# Autodesk Inventor assembly: Assembly1_TT
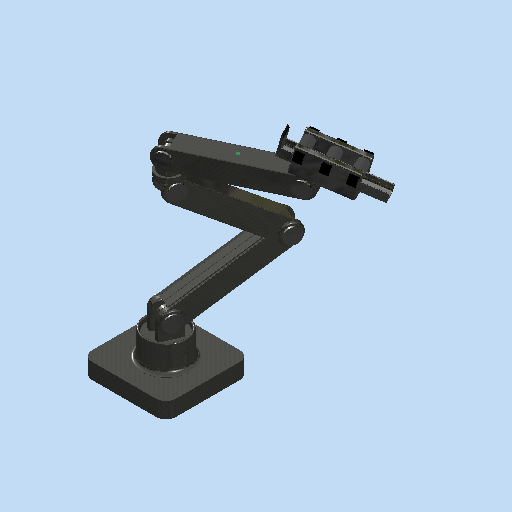
[picture p0: Inventor's stored thumbnail of the model, 512x512]
Saved by Autodesk Inventor 2027.1 (Build 311270010, 270A)
## iProperties
Created: 2026-08-27
Part Number: Assembly1_TT
Document SubType Name: Assembly
Designer: RIDDHIMAN
Author: RIDDHIMAN
## Documents named in this file (12)
- D:\ZINE ROUND 2\Assembly1_TT.iam
- D:\ZINE ROUND 2\HANDBASE2.ipt
- D:\ZINE ROUND 2\TT_ARM1.ipt
- D:\ZINE ROUND 2\TT_ARM12.ipt
- D:\ZINE ROUND 2\HANDBASE1.ipt
- D:\ZINE ROUND 2\joint1.ipt
- D:\ZINE ROUND 2\joint2.ipt
- D:\ZINE ROUND 2\JOINT BASE2.ipt
- D:\ZINE ROUND 2\JOINT BASE1.ipt
- D:\ZINE ROUND 2\SHOOTING GUN.ipt
- D:\ZINE ROUND 2\ROLLER SHAFT.ipt
- D:\ZINE ROUND 2\ROLLER.ipt
## Components (19 placed, 11 different names)
1. HANDBASE2:1 — Rotational:3
2. TT_ARM1:1 — Rotational:1, Rotational:2, Rigid:2
3. TT_ARM12:1 — Rotational:2, Rigid:1, Rigid:3, Rotational:4
4. HANDBASE1:1 — Rotational:1, Rotational:3
5. joint1:1 — Rigid:1
6. joint1:2 — Rigid:2
7. joint2:1 — Rigid:3
8. JOINT BASE2:1 — Rotational:5, Rotational:6
9. TT_ARM12:2 — Rotational:6, Rigid:4, Rotational:7
10. JOINT BASE1:1 — Rotational:4, Rotational:5
11. joint2:2 — Rigid:4
12. SHOOTING GUN:1 — Rotational:7, Rigid:5, Rigid:6, Rigid:7, Rigid:8
13. joint2:3 — Rigid:5
14. ROLLER SHAFT:1 — Rotational:8, Rigid:6
15. ROLLER:1 — Rotational:8
16. ROLLER SHAFT:2 — Rigid:7
17. ROLLER:2
18. ROLLER SHAFT:3 — Rigid:8
19. ROLLER:3
## Relationships (18: RevoluteJoint 10, WeldJoint 8)
- Rotational:1 [RevoluteJoint]: TT_ARM1:1 ↔ HANDBASE1:1
- Rotational:2 [RevoluteJoint]: TT_ARM1:1 ↔ TT_ARM12:1
- Rotational:3 [RevoluteJoint]: HANDBASE2:1 ↔ HANDBASE1:1
- Rigid:1 [WeldJoint]: TT_ARM12:1 ↔ joint1:1
- Rigid:2 [WeldJoint]: TT_ARM1:1 ↔ joint1:2
- Rigid:3 [WeldJoint]: TT_ARM12:1 ↔ joint2:1
- Rotational:4 [RevoluteJoint]: TT_ARM12:1 ↔ JOINT BASE1:1
- Rotational:5 [RevoluteJoint]: JOINT BASE2:1 ↔ JOINT BASE1:1
- Rotational:6 [RevoluteJoint]: JOINT BASE2:1 ↔ TT_ARM12:2
- Rigid:4 [WeldJoint]: TT_ARM12:2 ↔ joint2:2
- Rotational:7 [RevoluteJoint]: TT_ARM12:2 ↔ SHOOTING GUN:1
- Rigid:5 [WeldJoint]: SHOOTING GUN:1 ↔ joint2:3
- Rotational:8 [RevoluteJoint]: ROLLER SHAFT:1 ↔ ROLLER:1
- Rigid:6 [WeldJoint]: SHOOTING GUN:1 ↔ ROLLER SHAFT:1
- [RevoluteJoint]: ROLLER SHAFT:2 ↔ ROLLER:2
- Rigid:7 [WeldJoint]: SHOOTING GUN:1 ↔ ROLLER SHAFT:2
- [RevoluteJoint]: ROLLER SHAFT:3 ↔ ROLLER:3
- Rigid:8 [WeldJoint]: SHOOTING GUN:1 ↔ ROLLER SHAFT:3
## Named parameters: d45_d40 = 0 mm, d46_d41 = -167.424614 deg, d48_d40 = 0 mm, d49_d41 = -10.224258 deg
